# Autodesk Inventor assembly: mot_27_ass
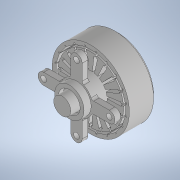
[picture p0: Inventor's stored thumbnail of the model, 180x180]
Saved by Autodesk Inventor 2020 (Build 240168000, 168)
## iProperties
Created: 2020-12-02
Part Number: mot_27_ass
Document SubType Name: Assembly
Designer: Shuang Peng
Author: Shuang Peng
## Documents named in this file (3)
- D:\projects-3\biped_tiny\hardware\mot_27_ass.iam
- D:\projects-3\biped_tiny\hardware\mot_27_2.ipt
- D:\projects-3\biped_tiny\hardware\mot_27_1.ipt
## Components (2 placed, 2 different names)
1. mot_27_2:1 — Insert:1, Angle:1
2. mot_27_1:1 — Insert:1, Angle:1
## Relationships (2: Insert 1, Angle 1)
- Insert:1: mot_27_2:1 ↔ mot_27_1:1
- Angle:1 (0 deg): mot_27_2:1 ↔ mot_27_1:1
